# Autodesk Inventor assembly: final-print
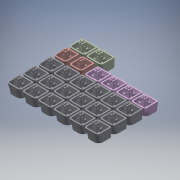
[picture p0: Inventor's stored thumbnail of the model, 180x180]
Saved by Autodesk Inventor 2018 (Build 220112000, 112)
## iProperties
Created: 2016-12-19
Part Number: final-print
Document SubType Name: Assembly
Designer: Cemra JC
Author: Cemra JC
## Documents named in this file (6)
- C:\Users\Jason Cemra\Documents\Logical Store\StenoToppers\stenotoppers\cherrymx\print-assemblies\final-print.iam
- C:\Users\Jason Cemra\Documents\Logical Store\StenoToppers\stenotoppers\cherrymx\stenotoppers\standard_cmx.ipt
- J:\The Files\The Software Files\Projects\stenotoppers\cherrymx\stenotoppers.ipt
- C:\Users\Jason Cemra\Documents\Logical Store\StenoToppers\stenotoppers\cherrymx\stenotoppers\smaller_cmx.ipt
- C:\Users\Jason Cemra\Documents\Logical Store\StenoToppers\stenotoppers\cherrymx\stenotoppers\larger_cmx.ipt
- C:\Users\Jason Cemra\Documents\Logical Store\StenoToppers\stenotoppers\cherrymx\stenotoppers\thumb_cmx.ipt
## Components (26 placed, 4 different names)
1. standard_cmx:1 — Mate:2
2. standard_cmx:5
3. standard_cmx:6
4. standard_cmx:7
5. standard_cmx:8
6. standard_cmx:9
7. standard_cmx:10
8. standard_cmx:11
9. standard_cmx:12
10. standard_cmx:13
11. standard_cmx:14
12. standard_cmx:15
13. standard_cmx:16
14. standard_cmx:17
15. standard_cmx:18
16. standard_cmx:19
17. standard_cmx:20
18. standard_cmx:21
19. smaller_cmx:2 — Mate:3
20. smaller_cmx:22
21. thumb_cmx:4 — Mate:1
22. thumb_cmx:23
23. thumb_cmx:24
24. thumb_cmx:25
25. larger_cmx:3 — Mate:4
26. larger_cmx:26
## Component patterns: (18 elements, first: standard_cmx:1), (2 elements, first: smaller_cmx:2), (4 elements, first: thumb_cmx:4), (2 elements, first: larger_cmx:3)
## Relationships (4: Mate 4)
- Mate:1: thumb_cmx:4
- Mate:2: standard_cmx:1
- Mate:3: smaller_cmx:2
- Mate:4: larger_cmx:3
